# Autodesk Inventor assembly: XCarriage
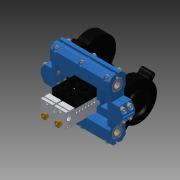
[picture p0: Inventor's stored thumbnail of the model, 180x180]
Saved by Autodesk Inventor 2015 SP1 (Build 190203100, 203)
## iProperties
Created: 2014-12-10
Part Number: XCarriage
Document SubType Name: Assembly
Designer: Jack
Mass: 269.669 g
Surface Area: 979.869 cm^2
Volume: 134.924 cm^3
Density: 1.99868 g/cm^3
Author: Jack
Title: X Carriage
## Documents named in this file (10)
- C:\Users\Jack\ownCloud\Projects\CrossBot\InventorModel\XAxis\XCarriage.iam
- C:\Users\Jack\ownCloud\Projects\CrossBot\InventorModel\HotEnds\E3DChimera\E3DChimera.iam
- C:\Users\Jack\ownCloud\Projects\CrossBot\InventorModel\Electronics\EndStops\EndStopOptical.ipt
- C:\Users\Jack\ownCloud\Projects\CrossBot\InventorModel\Hardware\Bearing\BearingLinear\BearingLinearLMU8.ipt
- C:\Users\Jack\ownCloud\Projects\CrossBot\InventorModel\XAxis\XCarriageBeltClipRound.ipt
- C:\Users\Jack\ownCloud\Projects\CrossBot\InventorModel\Electronics\Fans\FanRadial50mm.ipt
- C:\Users\Jack\ownCloud\Projects\CrossBot\InventorModel\XAxis\ChimeraXCarriage4.ipt
- C:\Users\Jack\ownCloud\Projects\CrossBot\InventorModel\Hardware\Nuts\Nut3.ipt
- C:\Users\Jack\ownCloud\Projects\CrossBot\InventorModel\Hardware\BoltWashers\BoltWasher3\BoltWasher3x16.iam
- C:\Users\Jack\ownCloud\Projects\CrossBot\InventorModel\Hardware\Bolts\SHCS\SHCS3\SHCS3x8.ipt
## Components (45 placed, 9 different names)
1. E3DChimera:1 [sub-assembly] — Mate:1, Mate:2, Mate:3
2. EndStopOptical:1 — Mate:81, Mate:82, Mate:83, Mate:84, Mate:85, Mate:86, Mate:87
3. BearingLinearLMU8:1 — Mate:7, Flush:1
4. BearingLinearLMU8:2 — Mate:6, Flush:4
5. BearingLinearLMU8:3 — Mate:5, Flush:3
6. BearingLinearLMU8:4 — Mate:4, Flush:2
7. XCarriageBeltClipRound:1 — Mate:14, Mate:16, Mate:18, Mate:41, Mate:43, Mate:53, Mate:56
8. XCarriageBeltClipRound:2 — Mate:15, Mate:17, Mate:19, Mate:42, Mate:44, Mate:54, Mate:55
9. XCarriageBeltClipRound:3 — Mate:8, Mate:11, Mate:12, Mate:45, Mate:47, Mate:49, Mate:51
10. XCarriageBeltClipRound:4 — Mate:9, Mate:10, Mate:13, Mate:46, Mate:48, Mate:50, Mate:52
11. FanRadial50mm:1 — Mate:22, Angle:1, Flush:5, Mate:23
12. FanRadial50mm:2 — Mate:21, Angle:2, Flush:5, Mate:24
13. ChimeraXCarriage4:1 — Mate:1, Mate:2, Mate:3, Mate:4, Mate:5, Mate:6, Mate:7, Flush:1, Flush:2, Flush:3, Flush:4, Mate:8, Mate:9, Mate:10, Mate:11, Mate:12, Mate:13, Mate:14, Mate:15, Mate:16, Mate:17, Mate:18, Mate:19, Mate:21, Mate:22, Angle:1, Angle:2, Mate:23, Mate:24, Mate:25, Mate:26, Angle:3, Mate:27, Mate:28, Angle:4, Mate:29, Mate:30, Angle:5, Mate:31, Mate:32, Angle:6, Mate:33, Mate:34, Mate:35, Mate:36, Mate:37, Angle:7, Mate:38, Angle:8, Mate:39, Mate:40, Angle:9, Angle:10, Mate:57, Mate:58, Mate:59, Mate:60, Mate:61, Mate:62, Mate:63, Mate:64, Mate:65, Mate:66, Mate:67, Mate:68, Angle:11, Angle:12, Angle:13, Angle:14, Angle:15, Angle:16, Mate:75, Mate:76, Mate:77, Mate:78, Mate:79, Mate:80, Mate:81, Mate:82, Mate:83, Mate:90, Mate:91, Angle:17, Angle:18
14. Nut3:15 — Mate:89, Mate:90, Angle:18
15. Nut3:16 — Mate:88, Mate:91, Angle:17
16. SHCS3x8:1 — Mate:84, Mate:85, Mate:89
17. SHCS3x8:2 — Mate:86, Mate:87, Mate:88
18. Nut3:14 — Mate:73, Angle:12, Mate:79
19. Nut3:13 — Mate:74, Angle:13, Mate:80
20. Nut3:12 — Mate:72, Angle:11, Mate:78
21. Nut3:10 — Mate:70, Angle:14, Mate:77
22. Nut3:11 — Mate:69, Angle:15, Mate:76
23. Nut3:9 — Mate:71, Angle:16, Mate:75
24. BoltWasher3x16:9 [sub-assembly] — Mate:59, Mate:61, Mate:73
25. BoltWasher3x16:10 [sub-assembly] — Mate:57, Mate:58, Mate:72
26. BoltWasher3x16:11 [sub-assembly] — Mate:60, Mate:62, Mate:74
27. BoltWasher3x16:12 [sub-assembly] — Mate:63, Mate:68, Mate:70
28. BoltWasher3x16:13 [sub-assembly] — Mate:64, Mate:67, Mate:69
29. BoltWasher3x16:14 [sub-assembly] — Mate:65, Mate:66, Mate:71
30. BoltWasher3x16:1 [sub-assembly] — Mate:42, Mate:55
31. BoltWasher3x16:2 [sub-assembly] — Mate:41, Mate:56
32. BoltWasher3x16:3 [sub-assembly] — Mate:43, Mate:53
33. BoltWasher3x16:4 [sub-assembly] — Mate:44, Mate:54
34. BoltWasher3x16:5 [sub-assembly] — Mate:45, Mate:49
35. BoltWasher3x16:6 [sub-assembly] — Mate:46, Mate:50
36. BoltWasher3x16:7 [sub-assembly] — Mate:47, Mate:51
37. BoltWasher3x16:8 [sub-assembly] — Mate:48, Mate:52
38. Nut3:1 — Mate:36, Mate:37, Angle:7
39. Nut3:2 — Mate:33, Mate:38, Angle:8
40. Nut3:3 — Mate:31, Mate:32, Angle:6
41. Nut3:4 — Mate:25, Mate:26, Angle:3
42. Nut3:5 — Mate:35, Mate:40, Angle:9
43. Nut3:6 — Mate:34, Mate:39, Angle:10
44. Nut3:7 — Mate:29, Mate:30, Angle:5
45. Nut3:8 — Mate:27, Mate:28, Angle:4
## Relationships (113: Mate 90, Angle 18, Flush 5)
- Mate:1: E3DChimera:1 ↔ ChimeraXCarriage4:1
- Mate:2: E3DChimera:1 ↔ ChimeraXCarriage4:1
- Mate:3: E3DChimera:1 ↔ ChimeraXCarriage4:1
- Mate:4: BearingLinearLMU8:4 ↔ ChimeraXCarriage4:1
- Mate:5: BearingLinearLMU8:3 ↔ ChimeraXCarriage4:1
- Mate:6: BearingLinearLMU8:2 ↔ ChimeraXCarriage4:1
- Mate:7: BearingLinearLMU8:1 ↔ ChimeraXCarriage4:1
- Flush:1: BearingLinearLMU8:1 ↔ ChimeraXCarriage4:1
- Flush:2: BearingLinearLMU8:4 ↔ ChimeraXCarriage4:1
- Flush:3: BearingLinearLMU8:3 ↔ ChimeraXCarriage4:1
- Flush:4: BearingLinearLMU8:2 ↔ ChimeraXCarriage4:1
- Mate:8: XCarriageBeltClipRound:3 ↔ ChimeraXCarriage4:1
- Mate:9: XCarriageBeltClipRound:4 ↔ ChimeraXCarriage4:1
- Mate:10: XCarriageBeltClipRound:4 ↔ ChimeraXCarriage4:1
- Mate:11: XCarriageBeltClipRound:3 ↔ ChimeraXCarriage4:1
- Mate:12: XCarriageBeltClipRound:3 ↔ ChimeraXCarriage4:1
- Mate:13: XCarriageBeltClipRound:4 ↔ ChimeraXCarriage4:1
- Mate:14: XCarriageBeltClipRound:1 ↔ ChimeraXCarriage4:1
- Mate:15: XCarriageBeltClipRound:2 ↔ ChimeraXCarriage4:1
- Mate:16: XCarriageBeltClipRound:1 ↔ ChimeraXCarriage4:1
- Mate:17: XCarriageBeltClipRound:2 ↔ ChimeraXCarriage4:1
- Mate:18: XCarriageBeltClipRound:1 ↔ ChimeraXCarriage4:1
- Mate:19: XCarriageBeltClipRound:2 ↔ ChimeraXCarriage4:1
- Mate:21: FanRadial50mm:2 ↔ ChimeraXCarriage4:1
- Mate:22: FanRadial50mm:1 ↔ ChimeraXCarriage4:1
- Angle:1 (180 deg): FanRadial50mm:1 ↔ ChimeraXCarriage4:1
- Angle:2 (180 deg): FanRadial50mm:2 ↔ ChimeraXCarriage4:1
- Flush:5: FanRadial50mm:1 ↔ FanRadial50mm:2
- Mate:23: FanRadial50mm:1 ↔ ChimeraXCarriage4:1
- Mate:24: FanRadial50mm:2 ↔ ChimeraXCarriage4:1
- Mate:25: ChimeraXCarriage4:1 ↔ Nut3:4
- Mate:26: ChimeraXCarriage4:1 ↔ Nut3:4
- Angle:3 (0 deg): ChimeraXCarriage4:1 ↔ Nut3:4
- Mate:27: ChimeraXCarriage4:1 ↔ Nut3:8
- Mate:28: ChimeraXCarriage4:1 ↔ Nut3:8
- Angle:4 (0 deg): ChimeraXCarriage4:1 ↔ Nut3:8
- Mate:29: ChimeraXCarriage4:1 ↔ Nut3:7
- Mate:30: ChimeraXCarriage4:1 ↔ Nut3:7
- Angle:5 (0 deg): ChimeraXCarriage4:1 ↔ Nut3:7
- Mate:31: ChimeraXCarriage4:1 ↔ Nut3:3
- Mate:32: ChimeraXCarriage4:1 ↔ Nut3:3
- Angle:6 (0 deg): ChimeraXCarriage4:1 ↔ Nut3:3
- Mate:33: ChimeraXCarriage4:1 ↔ Nut3:2
- Mate:34: ChimeraXCarriage4:1 ↔ Nut3:6
- Mate:35: ChimeraXCarriage4:1 ↔ Nut3:5
- Mate:36: ChimeraXCarriage4:1 ↔ Nut3:1
- Mate:37: ChimeraXCarriage4:1 ↔ Nut3:1
- Angle:7 (0 deg): ChimeraXCarriage4:1 ↔ Nut3:1
- Mate:38: ChimeraXCarriage4:1 ↔ Nut3:2
- Angle:8 (0 deg): ChimeraXCarriage4:1 ↔ Nut3:2
- Mate:39: ChimeraXCarriage4:1 ↔ Nut3:6
- Mate:40: ChimeraXCarriage4:1 ↔ Nut3:5
- Angle:9 (0 deg): ChimeraXCarriage4:1 ↔ Nut3:5
- Angle:10 (0 deg): ChimeraXCarriage4:1 ↔ Nut3:6
- Mate:41: XCarriageBeltClipRound:1 ↔ BoltWasher3x16:2
- Mate:42: XCarriageBeltClipRound:2 ↔ BoltWasher3x16:1
- Mate:43: XCarriageBeltClipRound:1 ↔ BoltWasher3x16:3
- Mate:44: XCarriageBeltClipRound:2 ↔ BoltWasher3x16:4
- Mate:45: XCarriageBeltClipRound:3 ↔ BoltWasher3x16:5
- Mate:46: XCarriageBeltClipRound:4 ↔ BoltWasher3x16:6
- Mate:47: XCarriageBeltClipRound:3 ↔ BoltWasher3x16:7
- Mate:48: XCarriageBeltClipRound:4 ↔ BoltWasher3x16:8
- Mate:49: XCarriageBeltClipRound:3 ↔ BoltWasher3x16:5
- Mate:50: XCarriageBeltClipRound:4 ↔ BoltWasher3x16:6
- Mate:51: XCarriageBeltClipRound:3 ↔ BoltWasher3x16:7
- Mate:52: XCarriageBeltClipRound:4 ↔ BoltWasher3x16:8
- Mate:53: XCarriageBeltClipRound:1 ↔ BoltWasher3x16:3
- Mate:54: XCarriageBeltClipRound:2 ↔ BoltWasher3x16:4
- Mate:55: XCarriageBeltClipRound:2 ↔ BoltWasher3x16:1
- Mate:56: XCarriageBeltClipRound:1 ↔ BoltWasher3x16:2
- Mate:57: ChimeraXCarriage4:1 ↔ BoltWasher3x16:10
- Mate:58: ChimeraXCarriage4:1 ↔ BoltWasher3x16:10
- Mate:59: ChimeraXCarriage4:1 ↔ BoltWasher3x16:9
- Mate:60: ChimeraXCarriage4:1 ↔ BoltWasher3x16:11
- Mate:61: ChimeraXCarriage4:1 ↔ BoltWasher3x16:9
- Mate:62: ChimeraXCarriage4:1 ↔ BoltWasher3x16:11
- Mate:63: ChimeraXCarriage4:1 ↔ BoltWasher3x16:12
- Mate:64: ChimeraXCarriage4:1 ↔ BoltWasher3x16:13
- Mate:65: ChimeraXCarriage4:1 ↔ BoltWasher3x16:14
- Mate:66: ChimeraXCarriage4:1 ↔ BoltWasher3x16:14
- Mate:67: ChimeraXCarriage4:1 ↔ BoltWasher3x16:13
- Mate:68: ChimeraXCarriage4:1 ↔ BoltWasher3x16:12
- Mate:69: Nut3:11 ↔ BoltWasher3x16:13
- Mate:70: Nut3:10 ↔ BoltWasher3x16:12
- Mate:71: Nut3:9 ↔ BoltWasher3x16:14
- Mate:72: Nut3:12 ↔ BoltWasher3x16:10
- Mate:73: Nut3:14 ↔ BoltWasher3x16:9
- Mate:74: Nut3:13 ↔ BoltWasher3x16:11
- Angle:11 (0 deg): ChimeraXCarriage4:1 ↔ Nut3:12
- Angle:12 (0 deg): ChimeraXCarriage4:1 ↔ Nut3:14
- Angle:13 (0 deg): ChimeraXCarriage4:1 ↔ Nut3:13
- Angle:14 (0 deg): ChimeraXCarriage4:1 ↔ Nut3:10
- Angle:15 (0 deg): ChimeraXCarriage4:1 ↔ Nut3:11
- Angle:16 (0 deg): ChimeraXCarriage4:1 ↔ Nut3:9
- Mate:75: ChimeraXCarriage4:1 ↔ Nut3:9
- Mate:76: ChimeraXCarriage4:1 ↔ Nut3:11
- Mate:77: ChimeraXCarriage4:1 ↔ Nut3:10
- Mate:78: ChimeraXCarriage4:1 ↔ Nut3:12
- Mate:79: ChimeraXCarriage4:1 ↔ Nut3:14
- Mate:80: ChimeraXCarriage4:1 ↔ Nut3:13
- Mate:81: EndStopOptical:1 ↔ ChimeraXCarriage4:1
- Mate:82: EndStopOptical:1 ↔ ChimeraXCarriage4:1
- Mate:83: EndStopOptical:1 ↔ ChimeraXCarriage4:1
- Mate:84: EndStopOptical:1 ↔ SHCS3x8:1
- Mate:85: EndStopOptical:1 ↔ SHCS3x8:1
- Mate:86: EndStopOptical:1 ↔ SHCS3x8:2
- Mate:87: EndStopOptical:1 ↔ SHCS3x8:2
- Mate:88: Nut3:16 ↔ SHCS3x8:2
- Mate:89: Nut3:15 ↔ SHCS3x8:1
- Mate:90: ChimeraXCarriage4:1 ↔ Nut3:15
- Mate:91: ChimeraXCarriage4:1 ↔ Nut3:16
- Angle:17 (0 deg): ChimeraXCarriage4:1 ↔ Nut3:16
- Angle:18 (0 deg): ChimeraXCarriage4:1 ↔ Nut3:15
